# Autodesk Inventor assembly: JewlArm
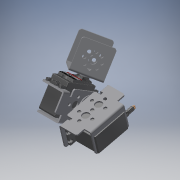
[picture p0: Inventor's stored thumbnail of the model, 180x180]
Saved by Autodesk Inventor 2017 (Build 210142000, 142)
## iProperties
Created: 2017-10-12
Part Number: JewlArm
Document SubType Name: Assembly
Designer: User
Author: User
## Documents named in this file (4)
- C:\Robotics\CAD\2017-18_CAD\JewlArm.iam
- C:\Robotics\CAD\COTSParts\Tetrix\Tetrix servo 180.ipt
- C:\Robotics\CAD\COTSParts\Tetrix\Tetrix bracket - single servo.ipt
- C:\Robotics\CAD\COTSParts\Tetrix\Tetrix channel 32mm.ipt
## Components (5 placed, 3 different names)
1. Tetrix servo 180:1 — Insert:5, Insert:7, Mate:3, Mate:4
2. Tetrix servo 180:2 — Insert:8, Insert:9, Insert:10, Insert:11
3. Tetrix bracket - single servo:1 — Insert:9, Insert:10
4. Tetrix bracket - single servo:2 — Insert:5, Mate:3, Insert:8, Insert:11
5. Tetrix channel 32mm:1 — Insert:7, Mate:4
## Relationships (8: Insert 6, Mate 2)
- Insert:5: Tetrix servo 180:1 ↔ Tetrix bracket - single servo:2
- Insert:7: Tetrix servo 180:1 ↔ Tetrix channel 32mm:1
- Mate:3: Tetrix servo 180:1 ↔ Tetrix bracket - single servo:2
- Mate:4: Tetrix servo 180:1 ↔ Tetrix channel 32mm:1
- Insert:8: Tetrix servo 180:2 ↔ Tetrix bracket - single servo:2
- Insert:9: Tetrix servo 180:2 ↔ Tetrix bracket - single servo:1
- Insert:10: Tetrix servo 180:2 ↔ Tetrix bracket - single servo:1
- Insert:11: Tetrix servo 180:2 ↔ Tetrix bracket - single servo:2
